# Autodesk Inventor assembly: Mark II Assembly
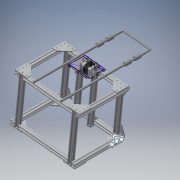
[picture p0: Inventor's stored thumbnail of the model, 180x180]
Saved by Autodesk Inventor 2016 (Build 200138000, 138)
## iProperties
Created: 2016-03-31
Part Number: Mark II Assembly
Document SubType Name: Assembly
Designer: Solomon
Author: Solomon
## Documents named in this file (11)
- C:\Users\Solomon\Documents\Inventor\SLA MK I\Mark II Assembly.iam
- C:\Users\Solomon\Documents\Inventor\SLA MK I\V Slot Part Files\Extrusions\vslot 20 x 20 v2 - 250mm.ipt
- C:\Users\Solomon\Documents\Inventor\SLA MK I\500mm M10.ipt
- C:\Users\Solomon\Documents\Inventor\SLA MK I\LM10UU.ipt
- C:\Users\Solomon\Documents\Inventor\SLA MK I\Motor pulley holder.ipt
- C:\Users\Solomon\Documents\Inventor\SLA MK I\140 mm m8.ipt
- C:\Users\Solomon\Documents\Inventor\SLA MK I\V Slot Part Files\Brackets and Joining Plates\5 Hole 90 Degree Bracket.ipt
- C:\Users\Solomon\Documents\Inventor\SLA MK I\V Slot Part Files\Brackets and Joining Plates\5 Hole T Joining Plate.ipt
- C:\Users\Solomon\Documents\Inventor\SLA MK I\V Slot Part Files\Brackets and Joining Plates\2 Hole Joining Strip Plate.ipt
- C:\Users\Solomon\Documents\Inventor\SLA MK I\V Slot Part Files\Brackets and Joining Plates\90 Degree Corner Connector.ipt
- C:\Users\Solomon\Documents\Inventor\stepper-motor-nema-17.snapshot.17\NEMA 17.ipt
## Components (39 placed, 10 different names)
1. vslot 20 x 20 v2 - 250mm:1 — Angle:1, Flush:1, Mate:1, Flush:2, Flush:3, Flush:4, Mate:2, Flush:15, Flush:16, Mate:8, Angle:10, Flush:31, Mate:21
2. vslot 20 x 20 v2 - 250mm:2 — Flush:5, Mate:3, Flush:6
3. vslot 20 x 20 v2 - 250mm:3 — Angle:1, Angle:2, Flush:3, Flush:4, Mate:2, Flush:5, Mate:3, Flush:6, Flush:24, Flush:42
4. vslot 20 x 20 v2 - 250mm:4 — Angle:2, Flush:1, Mate:1, Flush:2, Flush:23, Flush:28
5. vslot 20 x 20 v2 - 250mm:5 — Flush:13, Mate:7, Flush:14, Flush:19, Flush:20, Mate:10, Angle:12, Mate:20, Angle:14, Mate:23, Mate:24
6. vslot 20 x 20 v2 - 250mm:6 — Flush:18, Mate:9, Flush:21, Flush:22, Mate:11, Mate:15, Flush:29, Angle:15, Mate:22, Mate:25
7. vslot 20 x 20 v2 - 250mm:7 — Tangent:1, Tangent:2, Tangent:3, Tangent:4, Angle:7, Mate:12, Flush:25, Flush:26, Tangent:6, Flush:40, Flush:48, Flush:50
8. vslot 20 x 20 v2 - 250mm:8 — Flush:17, Flush:33, Flush:43, Flush:45, Mate:26, Flush:51, Flush:52, Mate:27, Mate:32, Mate:35
9. vslot 20 x 20 v2 - 250mm:10 — Flush:13, Mate:7, Flush:14, Flush:15, Flush:16, Mate:8, Mate:16, Flush:32, Mate:17, Flush:34, Angle:13, Flush:46
10. vslot 20 x 20 v2 - 250mm:11 — Flush:17, Flush:18, Mate:9, Flush:27, Mate:14, Angle:11, Flush:30, Flush:44
11. vslot 20 x 20 v2 - 250mm:13 — Flush:19, Flush:20, Mate:10, Angle:8, Flush:39, Flush:41, Flush:47
12. vslot 20 x 20 v2 - 250mm:14 — Flush:21, Flush:22, Mate:11, Mate:18, Mate:19, Flush:35, Flush:36, Flush:38, Flush:37, Flush:49
13. 500mm M10:2 — Flush:23, Tangent:1, Tangent:2, Angle:6, Insert:3, Insert:4
14. 500mm M10:3 — Flush:24, Tangent:3, Tangent:4, Angle:5, Insert:1, Insert:2, Tangent:5, Mate:13
15. LM10UU:1 — Angle:5, Insert:1
16. LM10UU:2 — Angle:6, Insert:3
17. LM10UU:3 — Insert:2
18. LM10UU:4 — Insert:4
19. Motor pulley holder:1 — Angle:7, Mate:12, Flush:25, Flush:26, Angle:19, Angle:22, Mate:36, Angle:23
20. 140 mm m8:1 — Angle:8, Tangent:5, Mate:13, Tangent:6
21. 5 Hole 90 Degree Bracket:1 — Flush:27, Flush:28, Mate:14
22. 5 Hole 90 Degree Bracket:2 — Angle:10, Mate:16, Flush:31, Flush:32
23. 5 Hole 90 Degree Bracket:4 — Angle:11, Mate:15, Flush:29, Flush:30, Angle:17
24. 5 Hole 90 Degree Bracket:5 — Angle:12, Mate:17, Flush:33, Flush:34, Angle:18
25. 5 Hole 90 Degree Bracket:6 — Mate:19, Flush:35, Flush:36
26. 5 Hole 90 Degree Bracket:7 — Mate:21, Flush:41, Flush:42
27. 5 Hole 90 Degree Bracket:8 — Mate:18, Flush:37, Flush:38, Angle:16
28. 5 Hole 90 Degree Bracket:9 — Mate:20, Flush:39, Flush:40
29. 5 Hole T Joining Plate:1 — Angle:13, Angle:19, Mate:24, Flush:47, Flush:48
30. 5 Hole T Joining Plate:2 — Angle:14, Angle:18, Flush:45, Flush:46, Mate:23
31. 5 Hole T Joining Plate:4 — Angle:15, Angle:17, Flush:43, Mate:22, Flush:44
32. 5 Hole T Joining Plate:5 — Angle:16, Flush:49, Flush:50, Mate:25
33. vslot 20 x 20 v2 - 250mm:15 — Mate:26, Flush:51, Angle:21, Mate:28, Mate:30, Flush:53, Mate:33
34. vslot 20 x 20 v2 - 250mm:16 — Flush:52, Mate:27, Angle:20, Mate:29, Mate:31, Mate:34, Flush:54
35. 2 Hole Joining Strip Plate 2 Hole Joining Strip Plate:1 — Angle:21, Mate:28, Mate:30
36. 2 Hole Joining Strip Plate 2 Hole Joining Strip Plate:2 — Angle:20, Mate:29, Mate:31
37. 90 Degree Corner Connector:1 — Mate:34, Flush:54, Mate:35
38. 90 Degree Corner Connector:2 — Flush:53, Mate:32, Mate:33
39. NEMA 17:1 — Angle:22, Mate:36, Angle:23
## Relationships (122: Flush 54, Mate 36, Angle 22, Tangent 6, Insert 4)
- Angle:1 (0 deg): vslot 20 x 20 v2 - 250mm:1 ↔ vslot 20 x 20 v2 - 250mm:3
- Angle:2 (0 deg): vslot 20 x 20 v2 - 250mm:3 ↔ vslot 20 x 20 v2 - 250mm:4
- Flush:1: vslot 20 x 20 v2 - 250mm:1 ↔ vslot 20 x 20 v2 - 250mm:4
- Mate:1: vslot 20 x 20 v2 - 250mm:1 ↔ vslot 20 x 20 v2 - 250mm:4
- Flush:2: vslot 20 x 20 v2 - 250mm:1 ↔ vslot 20 x 20 v2 - 250mm:4
- Flush:3: vslot 20 x 20 v2 - 250mm:1 ↔ vslot 20 x 20 v2 - 250mm:3
- Flush:4: vslot 20 x 20 v2 - 250mm:1 ↔ vslot 20 x 20 v2 - 250mm:3
- Mate:2: vslot 20 x 20 v2 - 250mm:1 ↔ vslot 20 x 20 v2 - 250mm:3
- Flush:5: vslot 20 x 20 v2 - 250mm:2 ↔ vslot 20 x 20 v2 - 250mm:3
- Mate:3: vslot 20 x 20 v2 - 250mm:2 ↔ vslot 20 x 20 v2 - 250mm:3
- Flush:6: vslot 20 x 20 v2 - 250mm:2 ↔ vslot 20 x 20 v2 - 250mm:3
- [Angle] (0 deg): vslot 20 x 20 v2 - 250mm:5 ↔ vslot 20 x 20 v2 - 250mm:7
- [Angle] (0 deg): vslot 20 x 20 v2 - 250mm:7 ↔ vslot 20 x 20 v2 - 250mm:8
- [Flush]: vslot 20 x 20 v2 - 250mm:5 ↔ vslot 20 x 20 v2 - 250mm:8
- [Mate]: vslot 20 x 20 v2 - 250mm:5 ↔ vslot 20 x 20 v2 - 250mm:8
- [Flush]: vslot 20 x 20 v2 - 250mm:5 ↔ vslot 20 x 20 v2 - 250mm:8
- [Flush]: vslot 20 x 20 v2 - 250mm:5 ↔ vslot 20 x 20 v2 - 250mm:7
- [Flush]: vslot 20 x 20 v2 - 250mm:5 ↔ vslot 20 x 20 v2 - 250mm:7
- [Mate]: vslot 20 x 20 v2 - 250mm:5 ↔ vslot 20 x 20 v2 - 250mm:7
- [Flush]: vslot 20 x 20 v2 - 250mm:6 ↔ vslot 20 x 20 v2 - 250mm:7
- [Mate]: vslot 20 x 20 v2 - 250mm:6 ↔ vslot 20 x 20 v2 - 250mm:7
- [Flush]: vslot 20 x 20 v2 - 250mm:6 ↔ vslot 20 x 20 v2 - 250mm:7
- Flush:13: vslot 20 x 20 v2 - 250mm:5 ↔ vslot 20 x 20 v2 - 250mm:10
- Mate:7: vslot 20 x 20 v2 - 250mm:5 ↔ vslot 20 x 20 v2 - 250mm:10
- Flush:14: vslot 20 x 20 v2 - 250mm:5 ↔ vslot 20 x 20 v2 - 250mm:10
- Flush:15: vslot 20 x 20 v2 - 250mm:1 ↔ vslot 20 x 20 v2 - 250mm:10
- Flush:16: vslot 20 x 20 v2 - 250mm:1 ↔ vslot 20 x 20 v2 - 250mm:10
- Mate:8: vslot 20 x 20 v2 - 250mm:1 ↔ vslot 20 x 20 v2 - 250mm:10
- Flush:17: vslot 20 x 20 v2 - 250mm:8 ↔ vslot 20 x 20 v2 - 250mm:11
- Flush:18: vslot 20 x 20 v2 - 250mm:6 ↔ vslot 20 x 20 v2 - 250mm:11
- Mate:9: vslot 20 x 20 v2 - 250mm:6 ↔ vslot 20 x 20 v2 - 250mm:11
- Flush:19: vslot 20 x 20 v2 - 250mm:5 ↔ vslot 20 x 20 v2 - 250mm:13
- Flush:20: vslot 20 x 20 v2 - 250mm:5 ↔ vslot 20 x 20 v2 - 250mm:13
- Mate:10: vslot 20 x 20 v2 - 250mm:5 ↔ vslot 20 x 20 v2 - 250mm:13
- Flush:21: vslot 20 x 20 v2 - 250mm:6 ↔ vslot 20 x 20 v2 - 250mm:14
- Flush:22: vslot 20 x 20 v2 - 250mm:6 ↔ vslot 20 x 20 v2 - 250mm:14
- Mate:11: vslot 20 x 20 v2 - 250mm:6 ↔ vslot 20 x 20 v2 - 250mm:14
- Flush:23: vslot 20 x 20 v2 - 250mm:4 ↔ 500mm M10:2
- Tangent:1: vslot 20 x 20 v2 - 250mm:7 ↔ 500mm M10:2
- Tangent:2 (50 mm): vslot 20 x 20 v2 - 250mm:7 ↔ 500mm M10:2
- Flush:24: vslot 20 x 20 v2 - 250mm:3 ↔ 500mm M10:3
- Tangent:3: vslot 20 x 20 v2 - 250mm:7 ↔ 500mm M10:3
- Tangent:4 (50 mm): vslot 20 x 20 v2 - 250mm:7 ↔ 500mm M10:3
- Angle:5 (0 deg): 500mm M10:3 ↔ LM10UU:1
- Angle:6 (0 deg): 500mm M10:2 ↔ LM10UU:2
- Insert:1 (100 mm): 500mm M10:3 ↔ LM10UU:1
- Insert:2 (50 mm): 500mm M10:3 ↔ LM10UU:3
- Insert:3 (100 mm): 500mm M10:2 ↔ LM10UU:2
- Insert:4 (50 mm): 500mm M10:2 ↔ LM10UU:4
- Angle:7 (0 deg): vslot 20 x 20 v2 - 250mm:7 ↔ Motor pulley holder:1
- Mate:12: vslot 20 x 20 v2 - 250mm:7 ↔ Motor pulley holder:1
- Flush:25: vslot 20 x 20 v2 - 250mm:7 ↔ Motor pulley holder:1
- Flush:26 (85 mm): vslot 20 x 20 v2 - 250mm:7 ↔ Motor pulley holder:1
- Angle:8 (0 deg): vslot 20 x 20 v2 - 250mm:13 ↔ 140 mm m8:1
- Tangent:5: 500mm M10:3 ↔ 140 mm m8:1
- Mate:13: 500mm M10:3 ↔ 140 mm m8:1
- Tangent:6 (-23 mm): vslot 20 x 20 v2 - 250mm:7 ↔ 140 mm m8:1
- Flush:27: vslot 20 x 20 v2 - 250mm:11 ↔ 5 Hole 90 Degree Bracket:1
- Flush:28: vslot 20 x 20 v2 - 250mm:4 ↔ 5 Hole 90 Degree Bracket:1
- Mate:14: vslot 20 x 20 v2 - 250mm:11 ↔ 5 Hole 90 Degree Bracket:1
- Angle:10 (0 deg): vslot 20 x 20 v2 - 250mm:1 ↔ 5 Hole 90 Degree Bracket:2
- Angle:11 (0 deg): vslot 20 x 20 v2 - 250mm:11 ↔ 5 Hole 90 Degree Bracket:4
- Mate:15: vslot 20 x 20 v2 - 250mm:6 ↔ 5 Hole 90 Degree Bracket:4
- Flush:29: vslot 20 x 20 v2 - 250mm:6 ↔ 5 Hole 90 Degree Bracket:4
- Flush:30: vslot 20 x 20 v2 - 250mm:11 ↔ 5 Hole 90 Degree Bracket:4
- Mate:16: vslot 20 x 20 v2 - 250mm:10 ↔ 5 Hole 90 Degree Bracket:2
- Flush:31: vslot 20 x 20 v2 - 250mm:1 ↔ 5 Hole 90 Degree Bracket:2
- Flush:32: vslot 20 x 20 v2 - 250mm:10 ↔ 5 Hole 90 Degree Bracket:2
- Angle:12 (0 deg): vslot 20 x 20 v2 - 250mm:5 ↔ 5 Hole 90 Degree Bracket:5
- Mate:17: vslot 20 x 20 v2 - 250mm:10 ↔ 5 Hole 90 Degree Bracket:5
- Flush:33: vslot 20 x 20 v2 - 250mm:8 ↔ 5 Hole 90 Degree Bracket:5
- Flush:34: vslot 20 x 20 v2 - 250mm:10 ↔ 5 Hole 90 Degree Bracket:5
- Mate:18: vslot 20 x 20 v2 - 250mm:14 ↔ 5 Hole 90 Degree Bracket:8
- Mate:19: vslot 20 x 20 v2 - 250mm:14 ↔ 5 Hole 90 Degree Bracket:6
- Mate:20: vslot 20 x 20 v2 - 250mm:5 ↔ 5 Hole 90 Degree Bracket:9
- Mate:21: vslot 20 x 20 v2 - 250mm:1 ↔ 5 Hole 90 Degree Bracket:7
- Flush:35: vslot 20 x 20 v2 - 250mm:14 ↔ 5 Hole 90 Degree Bracket:6
- Flush:36: vslot 20 x 20 v2 - 250mm:14 ↔ 5 Hole 90 Degree Bracket:6
- Flush:37: vslot 20 x 20 v2 - 250mm:14 ↔ 5 Hole 90 Degree Bracket:8
- Flush:38: vslot 20 x 20 v2 - 250mm:14 ↔ 5 Hole 90 Degree Bracket:8
- Flush:39: vslot 20 x 20 v2 - 250mm:13 ↔ 5 Hole 90 Degree Bracket:9
- Flush:40: vslot 20 x 20 v2 - 250mm:7 ↔ 5 Hole 90 Degree Bracket:9
- Flush:41: vslot 20 x 20 v2 - 250mm:13 ↔ 5 Hole 90 Degree Bracket:7
- Flush:42: vslot 20 x 20 v2 - 250mm:3 ↔ 5 Hole 90 Degree Bracket:7
- Angle:13 (0 deg): vslot 20 x 20 v2 - 250mm:10 ↔ 5 Hole T Joining Plate:1
- Angle:14 (0 deg): vslot 20 x 20 v2 - 250mm:5 ↔ 5 Hole T Joining Plate:2
- Angle:15 (0 deg): vslot 20 x 20 v2 - 250mm:6 ↔ 5 Hole T Joining Plate:4
- Angle:16 (0 deg): 5 Hole 90 Degree Bracket:8 ↔ 5 Hole T Joining Plate:5
- Angle:17 (0 deg): 5 Hole 90 Degree Bracket:4 ↔ 5 Hole T Joining Plate:4
- Angle:18 (0 deg): 5 Hole 90 Degree Bracket:5 ↔ 5 Hole T Joining Plate:2
- Angle:19 (0 deg): Motor pulley holder:1 ↔ 5 Hole T Joining Plate:1
- Flush:43: vslot 20 x 20 v2 - 250mm:8 ↔ 5 Hole T Joining Plate:4
- Mate:22: vslot 20 x 20 v2 - 250mm:6 ↔ 5 Hole T Joining Plate:4
- Flush:44: vslot 20 x 20 v2 - 250mm:11 ↔ 5 Hole T Joining Plate:4
- Flush:45: vslot 20 x 20 v2 - 250mm:8 ↔ 5 Hole T Joining Plate:2
- Flush:46: vslot 20 x 20 v2 - 250mm:10 ↔ 5 Hole T Joining Plate:2
- Mate:23: vslot 20 x 20 v2 - 250mm:5 ↔ 5 Hole T Joining Plate:2
- Mate:24: vslot 20 x 20 v2 - 250mm:5 ↔ 5 Hole T Joining Plate:1
- Flush:47: vslot 20 x 20 v2 - 250mm:13 ↔ 5 Hole T Joining Plate:1
- Flush:48: vslot 20 x 20 v2 - 250mm:7 ↔ 5 Hole T Joining Plate:1
- Flush:49: vslot 20 x 20 v2 - 250mm:14 ↔ 5 Hole T Joining Plate:5
- Flush:50: vslot 20 x 20 v2 - 250mm:7 ↔ 5 Hole T Joining Plate:5
- Mate:25: vslot 20 x 20 v2 - 250mm:6 ↔ 5 Hole T Joining Plate:5
- Mate:26: vslot 20 x 20 v2 - 250mm:8 ↔ vslot 20 x 20 v2 - 250mm:15
- Flush:51: vslot 20 x 20 v2 - 250mm:8 ↔ vslot 20 x 20 v2 - 250mm:15
- Flush:52: vslot 20 x 20 v2 - 250mm:8 ↔ vslot 20 x 20 v2 - 250mm:16
- Mate:27: vslot 20 x 20 v2 - 250mm:8 ↔ vslot 20 x 20 v2 - 250mm:16
- Angle:20 (0 deg): vslot 20 x 20 v2 - 250mm:16 ↔ 2 Hole Joining Strip Plate 2 Hole Joining Strip Plate:2
- Angle:21 (0 deg): vslot 20 x 20 v2 - 250mm:15 ↔ 2 Hole Joining Strip Plate 2 Hole Joining Strip Plate:1
- Mate:28: vslot 20 x 20 v2 - 250mm:15 ↔ 2 Hole Joining Strip Plate 2 Hole Joining Strip Plate:1
- Mate:29: vslot 20 x 20 v2 - 250mm:16 ↔ 2 Hole Joining Strip Plate 2 Hole Joining Strip Plate:2
- Mate:30: vslot 20 x 20 v2 - 250mm:15 ↔ 2 Hole Joining Strip Plate 2 Hole Joining Strip Plate:1
- Mate:31: vslot 20 x 20 v2 - 250mm:16 ↔ 2 Hole Joining Strip Plate 2 Hole Joining Strip Plate:2
- Flush:53: vslot 20 x 20 v2 - 250mm:15 ↔ 90 Degree Corner Connector:2
- Mate:32: vslot 20 x 20 v2 - 250mm:8 ↔ 90 Degree Corner Connector:2
- Mate:33: vslot 20 x 20 v2 - 250mm:15 ↔ 90 Degree Corner Connector:2
- Mate:34: vslot 20 x 20 v2 - 250mm:16 ↔ 90 Degree Corner Connector:1
- Flush:54: vslot 20 x 20 v2 - 250mm:16 ↔ 90 Degree Corner Connector:1
- Mate:35: vslot 20 x 20 v2 - 250mm:8 ↔ 90 Degree Corner Connector:1
- Angle:22 (0 deg): Motor pulley holder:1 ↔ NEMA 17:1
- Mate:36: Motor pulley holder:1 ↔ NEMA 17:1
- Angle:23 (0 deg): Motor pulley holder:1 ↔ NEMA 17:1
## Named parameters: d11_d2 = 0 mm, d12_d3 = 0 mm, d13_d4 = 0 mm, d14_d5 = 0 mm, d15_d6 = 0 mm, d16_d7 = 0 mm, d17_d8 = 0 mm, d18_d9 = 0 mm, d19_d10 = 0 mm, d20_d0 = 0 deg, d21_d1 = 0 deg
